# Autodesk Inventor assembly: Assembly1
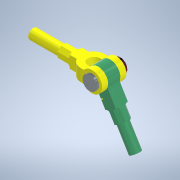
[picture p0: Inventor's stored thumbnail of the model, 180x180]
Saved by Autodesk Inventor 2021 (Build 250183000, 183)
## iProperties
Created: 2021-03-19
Part Number: Assembly1
Document SubType Name: Assembly
Designer: uriel
Author: uriel
## Documents named in this file (6)
- C:\Users\uriel\Documents\Escuela\LABORATORIO DISEÑO Y MANUFACTURA ASISTIDA POR COMPUTADORA\Practica 2\Assembly1.iam
- C:\Users\uriel\Documents\Escuela\LABORATORIO DISEÑO Y MANUFACTURA ASISTIDA POR COMPUTADORA\Practica 2\J Collar.ipt
- C:\Users\uriel\Documents\Escuela\LABORATORIO DISEÑO Y MANUFACTURA ASISTIDA POR COMPUTADORA\Practica 2\J Eye end.ipt
- C:\Users\uriel\Documents\Escuela\LABORATORIO DISEÑO Y MANUFACTURA ASISTIDA POR COMPUTADORA\Practica 2\J Fork end.ipt
- C:\Users\uriel\Documents\Escuela\LABORATORIO DISEÑO Y MANUFACTURA ASISTIDA POR COMPUTADORA\Practica 2\J Pasador.ipt
- C:\Users\uriel\Documents\Escuela\LABORATORIO DISEÑO Y MANUFACTURA ASISTIDA POR COMPUTADORA\Practica 2\J Perno.ipt
## Components (5 placed, 5 different names)
1. J Collar:1 — Mate:1, Mate:2, Mate:3, Mate:4
2. J Eye end:1 — Insert:1
3. J Fork end:1 — Insert:1, Insert:2
4. J Pasador:1 — Mate:3, Mate:4
5. J Perno:1 — Insert:2, Mate:1, Mate:2
## Relationships (6: Mate 4, Insert 2)
- Insert:1: J Eye end:1 ↔ J Fork end:1
- Insert:2: J Fork end:1 ↔ J Perno:1
- Mate:1: J Collar:1 ↔ J Perno:1
- Mate:2: J Collar:1 ↔ J Perno:1
- Mate:3: J Collar:1 ↔ J Pasador:1
- Mate:4 (36 mm): J Collar:1 ↔ J Pasador:1
